# Autodesk Inventor assembly: EndEff
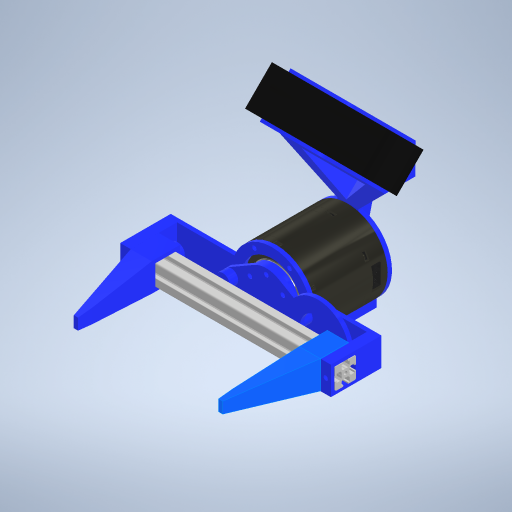
[picture p0: Inventor's stored thumbnail of the model, 512x512]
Saved by Autodesk Inventor 2024 (Build 280153000, 153)
## iProperties
Created: 2024-12-13
Part Number: EndEff
Document SubType Name: Assembly
Designer: hirek
Mass: 518.48 g
Surface Area: 1350.12 cm^2
Volume: 227.712 cm^3
Density: 2.27691 g/cm^3
Author: hirek
## Documents named in this file (9)
- E:\Documents\Inventor\CanAloha\EndEff.iam
- E:\Documents\Inventor\CanAloha\official\robStride00\robStride00.iam
- E:\Documents\Inventor\CanAloha\official\HFS3-1515\HFS3-1515-150.ipt
- E:\Documents\Inventor\CanAloha\myperts\endeff_3dp1.ipt
- E:\Documents\Inventor\CanAloha\myperts\endeff_3dp2.ipt
- E:\Documents\Inventor\CanAloha\myperts\endeff_3dp3.ipt
- E:\Documents\Inventor\CanAloha\myperts\endeff_3dp4.ipt
- E:\Documents\Inventor\CanAloha\official\camera.ipt
- E:\Documents\Inventor\CanAloha\official\camera_mount.ipt
## Components (10 placed, 8 different names)
1. robStride00:1 [sub-assembly] — 回転:1, 回転:2, 挿入:1
2. HFS3-1515-150:1 — メイト:1, メイト:2, メイト:3, メイト:4, メイト:5, メイト:6
3. endeff_3dp1:1 — 回転:1, 回転:2, メイト:1, メイト:2, 回転:7, メイト:7, 回転:8
4. endeff_3dp2:1 — 挿入:1, 回転:3, 回転:4
5. endeff_3dp3:2 — 回転:3, 回転:6
6. endeff_3dp3:3 — 回転:4, 回転:5
7. endeff_3dp4:1 — メイト:3, メイト:6, 回転:5
8. endeff_3dp4:2 — メイト:4, メイト:5, 回転:6
9. camera:1 — 回転:7, メイト:7
10. camera_mount:1 — 回転:8
## Relationships (16: RevoluteJoint 8, Mate 7, Insert 1)
- 回転:1 [RevoluteJoint]: robStride00:1 ↔ endeff_3dp1:1
- 回転:2 [RevoluteJoint]: robStride00:1 ↔ endeff_3dp1:1
- 挿入:1 [Insert]: robStride00:1 ↔ endeff_3dp2:1
- 回転:3 [RevoluteJoint]: endeff_3dp2:1 ↔ endeff_3dp3:2
- 回転:4 [RevoluteJoint]: endeff_3dp2:1 ↔ endeff_3dp3:3
- メイト:1 [Mate]: HFS3-1515-150:1 ↔ endeff_3dp1:1
- メイト:2 [Mate]: HFS3-1515-150:1 ↔ endeff_3dp1:1
- メイト:3 [Mate]: HFS3-1515-150:1 ↔ endeff_3dp4:1
- メイト:4 [Mate]: HFS3-1515-150:1 ↔ endeff_3dp4:2
- メイト:5 [Mate]: HFS3-1515-150:1 ↔ endeff_3dp4:2
- メイト:6 [Mate]: HFS3-1515-150:1 ↔ endeff_3dp4:1
- 回転:5 [RevoluteJoint]: endeff_3dp3:3 ↔ endeff_3dp4:1
- 回転:6 [RevoluteJoint]: endeff_3dp3:2 ↔ endeff_3dp4:2
- 回転:7 [RevoluteJoint]: endeff_3dp1:1 ↔ camera:1
- メイト:7 [Mate]: endeff_3dp1:1 ↔ camera:1
- 回転:8 [RevoluteJoint]: endeff_3dp1:1 ↔ camera_mount:1
